# Autodesk Inventor assembly: WelcoMount_wSwitch_v02
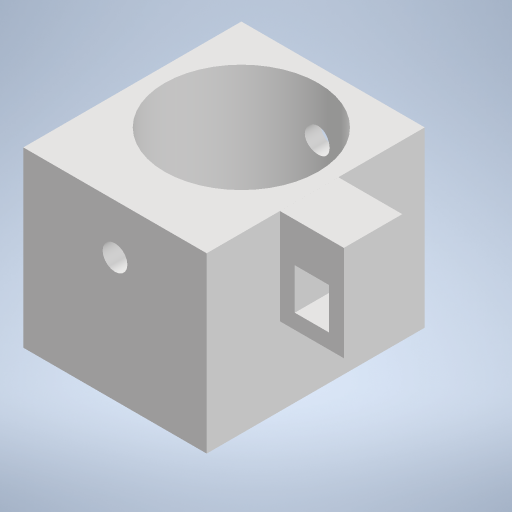
[picture p0: Inventor's stored thumbnail of the model, 512x512]
Saved by Autodesk Inventor 2023.5 (Build 275446000, 446)
## iProperties
Created: 2024-08-19
Part Number: WelcoMount_wSwitch_v02
Document SubType Name: Assembly
Designer: Akramilab
Author: Akramilab
## Documents named in this file (3)
- C:\Projects\Inventor\Touchscreen arena\Welco pump mount\WelcoMount_wSwitch_v02.iam
- C:\Projects\Inventor\Touchscreen arena\Welco pump mount\switch test v02b.ipt
- C:\Projects\Inventor\Touchscreen arena\Welco pump mount\welco mount v03b.ipt
## Components (2 placed, 2 different names)
1. switch test v02b:1 — Flush:1, Mate:1, Mate:2, Flush:2
2. welco mount v03b:1 — Flush:1, Mate:1, Mate:2, Flush:2
## Relationships (4: Flush 2, Mate 2)
- Flush:1: switch test v02b:1 ↔ welco mount v03b:1
- Mate:1: switch test v02b:1 ↔ welco mount v03b:1
- Mate:2: switch test v02b:1 ↔ welco mount v03b:1
- Flush:2: switch test v02b:1 ↔ welco mount v03b:1
